# Autodesk Inventor assembly: Assembly4
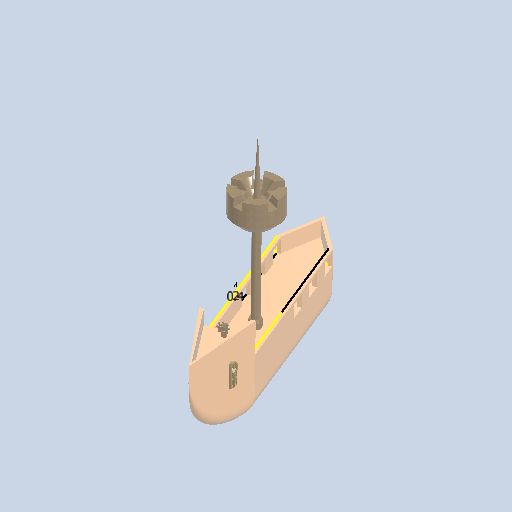
[picture p0: Inventor's stored thumbnail of the model, 512x512]
Saved by Autodesk Inventor 2024.1 (Build 281209000, 209)
## iProperties
Created: 2023-11-09
Part Number: Assembly4
Document SubType Name: Assembly
Designer: luvag
Author: luvag
## Documents named in this file (7)
- C:\Users\luvag\Desktop\Assembly4.iam
- C:\Users\luvag\Desktop\Madhup_Deck.ipt
- C:\Users\luvag\Desktop\Tower.ipt
- C:\Users\luvag\Desktop\bucket.ipt
- C:\Users\luvag\Desktop\trianglef.ipt
- C:\Users\luvag\Desktop\DOOROFSHIPCIRCLE.iam
- C:\Users\luvag\Desktop\Project Wheel.ipt
## Components (7 placed, 6 different names)
1. Madhup_Deck:1
2. Tower:1
3. bucket:1
4. trianglef:1
5. DOOROFSHIPCIRCLE:1 [sub-assembly]
6. DOOROFSHIPCIRCLE:2 [sub-assembly]
7. Project Wheel:1
## Relationships (8: Mate 8)
- [Mate]: Tower:1 ↔ trianglef:1
- [Mate]: bucket:1 ↔ trianglef:1
- [Mate]: Tower:1 ↔ bucket:1
- [Mate]: Tower:1 ↔ bucket:1
- [Mate]: Madhup_Deck:1 ↔ Tower:1
- [Mate]: Madhup_Deck:1 ↔ DOOROFSHIPCIRCLE:1
- [Mate]: Madhup_Deck:1 ↔ DOOROFSHIPCIRCLE:2
- [Mate]: Madhup_Deck:1 ↔ Project Wheel:1
